# Autodesk Inventor assembly: Body
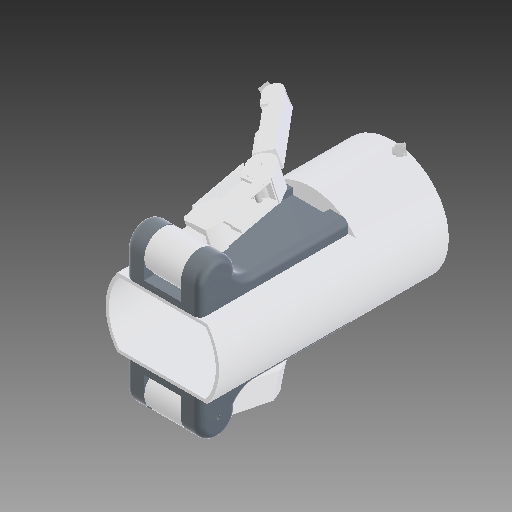
[picture p0: Inventor's stored thumbnail of the model, 512x512]
Saved by Autodesk Inventor 2017 SP1 (Build 210196100, 196)
## iProperties
Created: 2017-03-13
Part Number: Body
Document SubType Name: Assembly
Designer: zallen
Author: zallen
## Documents named in this file (3)
- C:\Users\Zach\Documents\GitHub\cr-laundry-robot\src\Body\Body.iam
- C:\Users\Zach\Documents\GitHub\cr-laundry-robot\src\Body\Chassis.ipt
- C:\Users\Zach\Documents\GitHub\cr-laundry-robot\src\Body\Arm Assembly\ArmAssembly.iam
## Components (3 placed, 2 different names)
1. Chassis:1 — Mate:6, Mate:9, Mate:11, Mate:12, Mate:13
2. ArmAssembly:1 [sub-assembly] — Mate:6, Mate:13, Mate:14
3. ArmAssembly:2 [sub-assembly] — Mate:9, Mate:11, Mate:12, Mate:14
## Relationships (6: Mate 6)
- Mate:6: Chassis:1 ↔ ArmAssembly:1
- Mate:9: Chassis:1 ↔ ArmAssembly:2
- Mate:11: Chassis:1 ↔ ArmAssembly:2
- Mate:12: Chassis:1 ↔ ArmAssembly:2
- Mate:13: Chassis:1 ↔ ArmAssembly:1
- Mate:14: ArmAssembly:1 ↔ ArmAssembly:2
